# Autodesk Inventor assembly: Assembly1
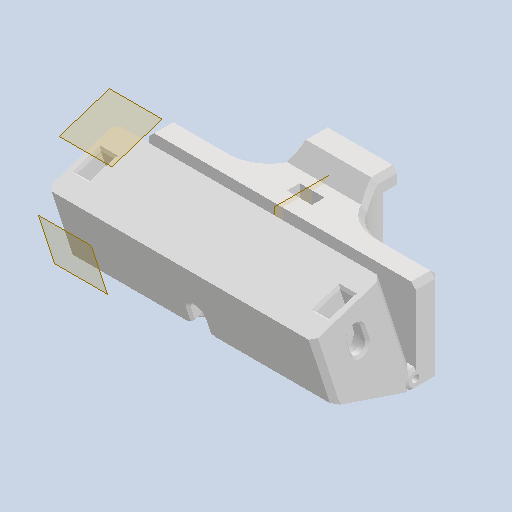
[picture p0: Inventor's stored thumbnail of the model, 512x512]
Saved by Autodesk Inventor 2022 (Build 260153000, 153)
## iProperties
Created: 2020-04-28
Part Number: Assembly1
Document SubType Name: Assembly
Designer: Daniel
Author: Daniel
## Documents named in this file (3)
- E:\OneDrive - Imperial College London\DragonVision_DanielKo\Instrumentation\Ephys_rig_2021\Projector_swing v2\swing_assembly.iam
- E:\OneDrive - Imperial College London\DragonVision_DanielKo\Instrumentation\Ephys_rig_2021\Projector_swing v2\swing.ipt
- E:\OneDrive - Imperial College London\DragonVision_DanielKo\Instrumentation\Ephys_rig_2021\Projector_swing v2\anchor.ipt
## Components (2 placed, 2 different names)
1. swing:1 — Flush:1, Mate:1, Angle:1
2. anchor:1 — Flush:1, Mate:1, Angle:1
## Relationships (3: Flush 1, Mate 1, Angle 1)
- Flush:1: swing:1 ↔ anchor:1
- Mate:1: swing:1 ↔ anchor:1
- Angle:1 (162 deg): swing:1 ↔ anchor:1
